# Autodesk Inventor assembly: Assembly1
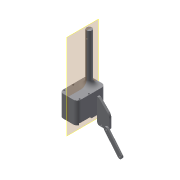
[picture p0: Inventor's stored thumbnail of the model, 180x180]
Saved by Autodesk Inventor 2018 (Build 220112000, 112)
## iProperties
Created: 2018-05-25
Part Number: Assembly1
Document SubType Name: Assembly
Designer: Bardo91
Author: Bardo91
## Documents named in this file (3)
- E:\programming\hecatonquiros\cad_models\tools\gripper\serial_model_0dof\gripper_2\Assembly1.iam
- E:\programming\hecatonquiros\cad_models\tools\gripper\serial_model_0dof\core_attachment.ipt
- E:\programming\hecatonquiros\cad_models\tools\gripper\serial_model_0dof\gripper_2\bar1.ipt
## Components (2 placed, 2 different names)
1. core_attachment:1 — Mate:1, Mate:2
2. bar1:1 — Mate:1, Mate:2
## Relationships (2: Mate 2)
- Mate:1: core_attachment:1 ↔ bar1:1
- Mate:2: core_attachment:1 ↔ bar1:1
